# Autodesk Inventor assembly: lightweight_bearing_MIR
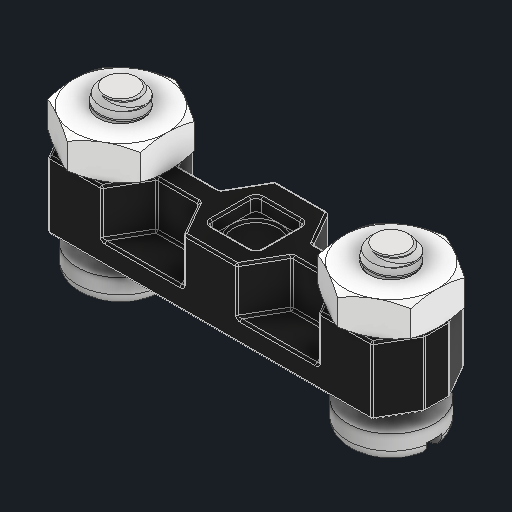
[picture p0: Inventor's stored thumbnail of the model, 512x512]
Saved by Autodesk Inventor 2024 (Build 280153000, 153)
## iProperties
Created: 2023-10-05
Part Number: lightweight_bearing_MIR
Document SubType Name: Assembly
Designer: Averey Ku
Author: Averey Ku
## Documents named in this file (5)
- D:\vex_robotics\hardware\cad\goated_v0.1\chassis\mirrored_parts\lightweight_bearing_MIR.iam
- D:\vex_robotics\hardware\cad\goated_v0.1\chassis\mirrored_parts\Bearing Flat Low Profile_MIR.ipt
- D:\vex_robotics\hardware\cad\goated_v0.1\chassis\mirrored_parts\Nylon Screw Pan-Head .500_MIR.ipt
- D:\vex_robotics\hardware\cad\VEX-CAD-Inventor-1.41\Structure\Hardware\Nut Nylon\Nut Nylon - White.ipt
- D:\vex_robotics\hardware\cad\VEX-CAD-Inventor-1.41\Structure\Hardware\Nut Nylon.ipt
## Components (5 placed, 3 different names)
1. Bearing Flat Low Profile_MIR:1 — Insert:1, Insert:2, Insert:3, Insert:4
2. Nylon Screw Pan-Head .500_MIR:1 — Insert:1
3. Nylon Screw Pan-Head .500_MIR:2 — Insert:2
4. Nut Nylon - White:1 — Insert:3
5. Nut Nylon - White:2 — Insert:4
## Relationships (4: Insert 4)
- Insert:1 (1.5875 mm): Bearing Flat Low Profile_MIR:1 ↔ Nylon Screw Pan-Head .500_MIR:1
- Insert:2 (1.5875 mm): Bearing Flat Low Profile_MIR:1 ↔ Nylon Screw Pan-Head .500_MIR:2
- Insert:3 (1.27 mm): Bearing Flat Low Profile_MIR:1 ↔ Nut Nylon - White:1
- Insert:4 (1.27 mm): Bearing Flat Low Profile_MIR:1 ↔ Nut Nylon - White:2
